# Autodesk Inventor assembly: Claw_1
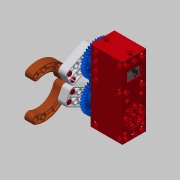
[picture p0: Inventor's stored thumbnail of the model, 180x180]
Saved by Autodesk Inventor 2019.3 (Build 233278000, 278)
## iProperties
Created: 2019-03-18
Part Number: Claw_1
Document SubType Name: Assembly
Designer: Varga Daniel
Author: Varga Daniel
## Documents named in this file (8)
- C:\!_Dani\!_cloud\OneDrive\!_munka\Revolution\RevvyDemoKit\Structural parts\Test assemblies\Claw_small_3.iam
- C:\!_Dani\!_cloud\OneDrive\!_munka\Revolution\RevvyDemoKit\Structural parts\Connetor Pins\CP1+x1+\CP1x1.ipt
- C:\!_Dani\!_cloud\OneDrive\!_munka\Revolution\RevvyDemoKit\Structural parts\Gears\G40.ipt
- C:\!_Dani\!_cloud\OneDrive\!_munka\Revolution\RevvyDemoKit\Structural parts\Demo parts\Motor\Inventor imported\motor.iam
- C:\!_Dani\!_cloud\OneDrive\!_munka\Revolution\RevvyDemoKit\Structural parts\Axles\AXp2p.ipt
- C:\!_Dani\!_cloud\OneDrive\!_munka\Revolution\RevvyDemoKit\Structural parts\Beams\Straight Beams\S2+x2\S4x2.ipt
- C:\!_Dani\!_cloud\OneDrive\!_munka\Revolution\RevvyDemoKit\Structural parts\Beams\Curved beams\CB4H.ipt
- C:\!_Dani\!_cloud\OneDrive\!_munka\Revolution\RevvyDemoKit\Structural parts\Connetor Pins\CP1+x1+\CP2x1.ipt
## Components (17 placed, 7 different names)
1. CB4H:1 — Insert:14, Insert:15
2. G40:1 — Mate:6, Angle:1, Rotation:1, Insert:16, Insert:17, Insert:23
3. motor:1 [sub-assembly] — Mate:1, Flush:1, Mate:2, Insert:5, Mate:6, Angle:2
4. AXp2p:1 — Mate:3, Mate:4, Mate:5, Insert:5
5. G40:2 — Mate:3, Mate:4, Mate:5, Angle:1, Angle:2, Rotation:1, Insert:19, Insert:20
6. CB4H:2 — Insert:10, Insert:11
7. S4x2:1 — Insert:8, Insert:9, Insert:18, Mate:7
8. S4x2:2 — Insert:12, Insert:13, Insert:21, Insert:22
9. CP1x1:4 — Insert:8, Insert:10
10. CP1x1:5 — Insert:9, Insert:11
11. CP1x1:6 — Insert:12, Insert:14
12. CP1x1:7 — Insert:13, Insert:15
13. CP2x1:2 — Insert:17, Mate:7
14. CP1x1:8 — Insert:16, Insert:18
15. CP1x1:9 — Insert:19, Insert:21
16. CP1x1:10 — Insert:20, Insert:22
17. CP1x1:11 — Insert:23
## Relationships (28: Insert 17, Mate 7, Angle 2, Flush 1, RelateRotation 1)
- Mate:1: motor:1
- Flush:1: motor:1
- Mate:2: motor:1
- Mate:3: AXp2p:1 ↔ G40:2
- Mate:4: AXp2p:1 ↔ G40:2
- Mate:5: AXp2p:1 ↔ G40:2
- Insert:5: motor:1 ↔ AXp2p:1
- Mate:6: G40:1 ↔ motor:1
- Angle:1 (0 deg): G40:1 ↔ G40:2
- Angle:2 (0 deg): motor:1 ↔ G40:2
- Insert:8: S4x2:1 ↔ CP1x1:4
- Insert:9: S4x2:1 ↔ CP1x1:5
- Insert:10: CB4H:2 ↔ CP1x1:4
- Insert:11: CB4H:2 ↔ CP1x1:5
- Insert:12: S4x2:2 ↔ CP1x1:6
- Insert:13: S4x2:2 ↔ CP1x1:7
- Insert:14: CB4H:1 ↔ CP1x1:6
- Insert:15: CB4H:1 ↔ CP1x1:7
- Rotation:1 [RelateRotation] (1 ul): G40:1 ↔ G40:2
- Insert:16: G40:1 ↔ CP1x1:8
- Insert:17: G40:1 ↔ CP2x1:2
- Insert:18: S4x2:1 ↔ CP1x1:8
- Mate:7: S4x2:1 ↔ CP2x1:2
- Insert:19: G40:2 ↔ CP1x1:9
- Insert:20: G40:2 ↔ CP1x1:10
- Insert:21: S4x2:2 ↔ CP1x1:9
- Insert:22: S4x2:2 ↔ CP1x1:10
- Insert:23: G40:1 ↔ CP1x1:11
